# Autodesk Inventor assembly: standoff
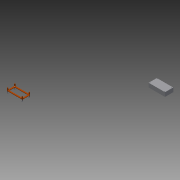
[picture p0: Inventor's stored thumbnail of the model, 180x180]
Saved by Autodesk Inventor 2014 (Build 180170000, 170)
## iProperties
Created: 2013-10-14
Part Number: standoff
Document SubType Name: Assembly
Designer: employee
Author: employee
## Documents named in this file (4)
- \\GRISTLE\speco\GitHub\ConceptFORGE\Wally\standoff.iam
- \\GRISTLE\speco\GitHub\ConceptFORGE\Wally\standoff.ipt
- \\GRISTLE\speco\GitHub\ConceptFORGE\Wally\M3x16.ipt
- \\GRISTLE\speco\GitHub\ConceptFORGE\Wally\electronics.ipt
## Components (6 placed, 3 different names)
1. standoff:1 — Insert:1, Insert:2, Insert:3, Insert:4, Insert:5, Mate:1
2. Forged Socket Head Cap Screw - Metric M3x0.5 x 16:1 — Insert:1
3. Forged Socket Head Cap Screw - Metric M3x0.5 x 16:2 — Insert:3
4. Forged Socket Head Cap Screw - Metric M3x0.5 x 16:3 — Insert:2
5. Forged Socket Head Cap Screw - Metric M3x0.5 x 16:4 — Insert:4
6. electronics:1 — Insert:5, Mate:1
## Relationships (6: Insert 5, Mate 1)
- Insert:1 (9.5 mm): standoff:1 ↔ Forged Socket Head Cap Screw - Metric M3x0.5 x 16:1
- Insert:2 (9.5 mm): standoff:1 ↔ Forged Socket Head Cap Screw - Metric M3x0.5 x 16:3
- Insert:3 (9.5 mm): standoff:1 ↔ Forged Socket Head Cap Screw - Metric M3x0.5 x 16:2
- Insert:4 (9.5 mm): standoff:1 ↔ Forged Socket Head Cap Screw - Metric M3x0.5 x 16:4
- Insert:5: standoff:1 ↔ electronics:1
- Mate:1: standoff:1 ↔ electronics:1
